# Autodesk Inventor assembly: BaseSlider
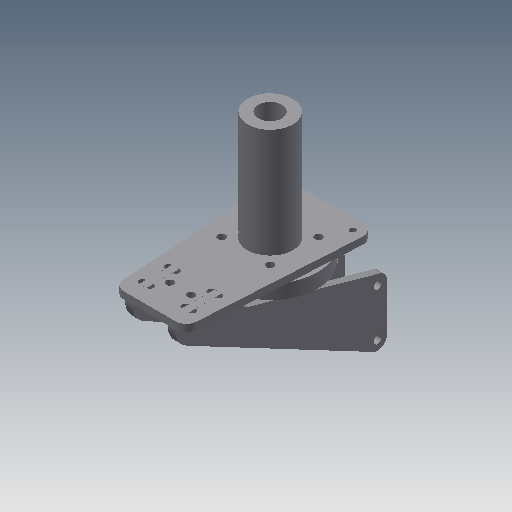
[picture p0: Inventor's stored thumbnail of the model, 512x512]
Saved by Autodesk Inventor 2019.4 (Build 234330000, 330)
## iProperties
Created: 2019-07-02
Part Number: BaseSlider
Document SubType Name: Assembly
Designer: AzLIer
Author: AzLIer
## Documents named in this file (5)
- E:\ロボ研\キャチロボ\キャチロボ2019\アーム2019\BaseSlider.iam
- E:\ロボ研\キャチロボ\キャチロボ2019\アーム2019\NB_SMF10WW.ipt
- E:\ロボ研\キャチロボ\キャチロボ2019\アーム2019\BaseSliderMount.ipt
- E:\ロボ研\キャチロボ\キャチロボ2019\アーム2019\BaseSliderSupport.ipt
- E:\ロボ研\キャチロボ\キャチロボ2019\アーム2019\tip3.ipt
## Components (6 placed, 4 different names)
1. NB_SMF10WW:1
2. BaseSliderMount:1
3. BaseSliderSupport:1
4. BaseSliderSupport:2
5. tip3:1
6. tip3:2
## Relationships (6: WeldJoint 4, RevoluteJoint 2)
- [RevoluteJoint]: NB_SMF10WW:1 ↔ BaseSliderMount:1
- [RevoluteJoint]: NB_SMF10WW:1 ↔ BaseSliderMount:1
- [WeldJoint]: BaseSliderSupport:1 ↔ tip3:1
- [WeldJoint]: BaseSliderSupport:2 ↔ tip3:2
- [WeldJoint]: BaseSliderMount:1 ↔ BaseSliderSupport:1
- [WeldJoint]: BaseSliderMount:1 ↔ BaseSliderSupport:2
